# Autodesk Inventor assembly: Lifting Part
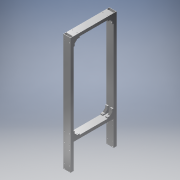
[picture p0: Inventor's stored thumbnail of the model, 180x180]
Saved by Autodesk Inventor 2019.4 (Build 234330000, 330)
## iProperties
Created: 2020-01-10
Part Number: Lifting Part
Document SubType Name: Assembly
Designer: Mark
Mass: 3786.5 g
Surface Area: 8769.78 cm^2
Volume: 1402.41 cm^3
Density: 2.7 g/cm^3
Author: Mark
## Documents named in this file (5)
- C:\Users\Mark\Desktop\7738 Helion Engineering\7738-2020\Elevator Mechanism\Lifting Part.iam
- C:\Users\Mark\Desktop\7738 Helion Engineering\7738-2020\Elevator Mechanism\Sliding Extrusions.ipt
- C:\Users\Mark\Desktop\7738 Helion Engineering\7738-2020\Elevator Mechanism\Middle Bar.ipt
- C:\Users\Mark\Desktop\7738 Helion Engineering\7738-2020\Elevator Mechanism\Standard Bracing.ipt
- C:\Users\Mark\Desktop\7738 Helion Engineering\7738-2020\Elevator Mechanism\Giant PC Plate.ipt
## Components (13 placed, 4 different names)
1. Sliding Extrusions:1 — Mate:1, Flush:1, Flush:2, Mate:2, Flush:3, Flush:4, Mate:9, Mate:11, Mate:15, Mate:16
2. Sliding Extrusions:2 — Mate:1, Flush:1, Flush:2, Mate:3, Flush:5, Flush:6, Mate:4, Mate:6, Mate:13, Mate:18, Flush:15, Flush:16
3. Middle Bar:1 — Mate:2, Flush:3, Flush:4, Flush:7, Mate:5, Flush:8, Mate:7, Mate:8, Flush:9, Flush:10, Mate:10
4. Middle Bar:2 — Mate:3, Flush:5, Flush:6, Mate:12, Flush:11, Mate:14, Flush:12, Flush:13, Mate:17, Mate:19, Flush:14, Mate:20
5. Standard Bracing:1 — Mate:12, Flush:11, Mate:13
6. Standard Bracing:2 — Flush:10, Mate:10, Mate:11
7. Standard Bracing:3 — Mate:8, Mate:9, Flush:9
8. Standard Bracing:4 — Flush:7, Mate:4, Mate:5
9. Standard Bracing:5 — Flush:8, Mate:6, Mate:7
10. Standard Bracing:6 — Flush:13, Mate:16, Mate:17
11. Standard Bracing:7 — Mate:18, Mate:19, Flush:14
12. Standard Bracing:8 — Mate:14, Mate:15, Flush:12
13. Giant PC Plate:1 — Mate:20, Flush:15, Flush:16
## Relationships (36: Mate 20, Flush 16)
- Mate:1 (333 mm): Sliding Extrusions:1 ↔ Sliding Extrusions:2
- Flush:1: Sliding Extrusions:1 ↔ Sliding Extrusions:2
- Flush:2: Sliding Extrusions:1 ↔ Sliding Extrusions:2
- Mate:2 (0.25 mm): Sliding Extrusions:1 ↔ Middle Bar:1
- Flush:3: Sliding Extrusions:1 ↔ Middle Bar:1
- Flush:4 (210 mm): Sliding Extrusions:1 ↔ Middle Bar:1
- Mate:3 (0.25 mm): Sliding Extrusions:2 ↔ Middle Bar:2
- Flush:5: Sliding Extrusions:2 ↔ Middle Bar:2
- Flush:6: Sliding Extrusions:2 ↔ Middle Bar:2
- Flush:7: Middle Bar:1 ↔ Standard Bracing:4
- Mate:4: Sliding Extrusions:2 ↔ Standard Bracing:4
- Mate:5: Middle Bar:1 ↔ Standard Bracing:4
- Flush:8: Middle Bar:1 ↔ Standard Bracing:5
- Mate:6: Sliding Extrusions:2 ↔ Standard Bracing:5
- Mate:7: Middle Bar:1 ↔ Standard Bracing:5
- Mate:8: Middle Bar:1 ↔ Standard Bracing:3
- Mate:9: Sliding Extrusions:1 ↔ Standard Bracing:3
- Flush:9: Middle Bar:1 ↔ Standard Bracing:3
- Flush:10: Middle Bar:1 ↔ Standard Bracing:2
- Mate:10: Middle Bar:1 ↔ Standard Bracing:2
- Mate:11: Sliding Extrusions:1 ↔ Standard Bracing:2
- Mate:12: Middle Bar:2 ↔ Standard Bracing:1
- Flush:11: Middle Bar:2 ↔ Standard Bracing:1
- Mate:13: Sliding Extrusions:2 ↔ Standard Bracing:1
- Mate:14: Middle Bar:2 ↔ Standard Bracing:8
- Mate:15: Sliding Extrusions:1 ↔ Standard Bracing:8
- Flush:12: Middle Bar:2 ↔ Standard Bracing:8
- Flush:13: Middle Bar:2 ↔ Standard Bracing:6
- Mate:16: Sliding Extrusions:1 ↔ Standard Bracing:6
- Mate:17: Middle Bar:2 ↔ Standard Bracing:6
- Mate:18: Sliding Extrusions:2 ↔ Standard Bracing:7
- Mate:19: Middle Bar:2 ↔ Standard Bracing:7
- Flush:14: Middle Bar:2 ↔ Standard Bracing:7
- Mate:20: Middle Bar:2 ↔ Giant PC Plate:1
- Flush:15: Sliding Extrusions:2 ↔ Giant PC Plate:1
- Flush:16: Sliding Extrusions:2 ↔ Giant PC Plate:1
